# Autodesk Inventor assembly: Fin assy test
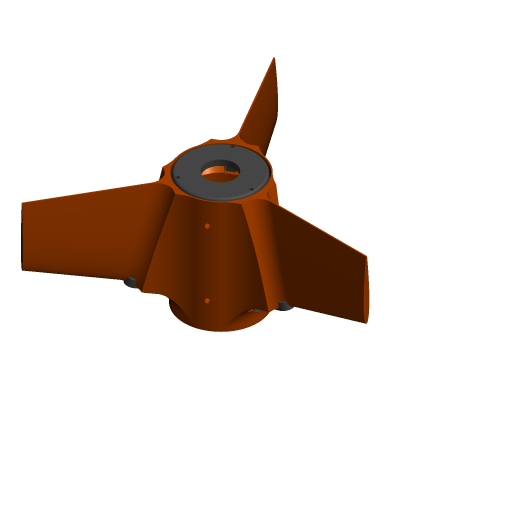
[picture p0: Inventor's stored thumbnail of the model, 512x512]
Saved by Autodesk Inventor 2024 (Build 280153000, 153)
## iProperties
Part Number: Fin assy test
Document SubType Name: Assembly
Designer: Jamie
Author: Jamie
## Documents named in this file (4)
- C:\Users\Jamie\Documents\Uni\DARE\Scrambler-2-CAD\Autodesk\Fin assy test.iam
- C:\Users\Jamie\Documents\Uni\DARE\Scrambler-2-CAD\Autodesk\Bigger fins with camera.ipt
- C:\Users\Jamie\Documents\Uni\DARE\Scrambler-2-CAD\Autodesk\Camera retention.ipt
- C:\Users\Jamie\Documents\Uni\DARE\Scrambler-2-CAD\Autodesk\Engine retention.ipt
## Components (5 placed, 3 different names)
1. Bigger fins with camera:1 — Mate:1, Mate:2, Mate:3
2. Engine retention:1 — Mate:3
3. Camera retention:1 — Mate:1, Mate:2
4. Camera retention:2
5. Camera retention:3
## Component patterns: (3 elements, first: Camera retention:1)
## Relationships (3: Mate 3)
- Mate:1: Bigger fins with camera:1 ↔ Camera retention:1
- Mate:2: Bigger fins with camera:1 ↔ Camera retention:1
- Mate:3: Bigger fins with camera:1 ↔ Engine retention:1
